# Autodesk Inventor assembly: Z Rail Right
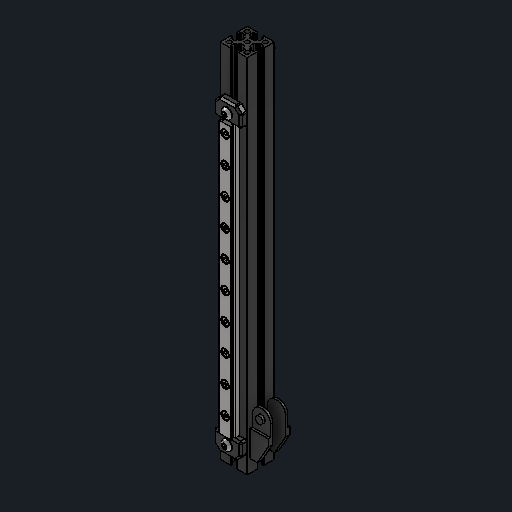
[picture p0: Inventor's stored thumbnail of the model, 512x512]
Saved by Autodesk Inventor 2026.1 (Build 301233020, 233B)
## iProperties
Created: 2025-05-11
Part Number: Z Rail Right
Document SubType Name: Assembly
Designer: Joshua Eah
Author: Joshua Eah
## Documents named in this file (9)
- C:\Users\JoshuaEah\Documents\GitHub\Voron-0\CAD\Z Axis\Z Extrusion Right.iam
- Z Extrusion Right.iam
- C:\Users\JoshuaEah\Documents\GitHub\Voron-0\CAD\Frame\Parts\1515_200mm - C.ipt
- C:\Users\JoshuaEah\Documents\GitHub\Voron-0\CAD\Hardware\M3x6 BHCS.ipt
- C:\Users\JoshuaEah\Documents\GitHub\Voron-0\CAD\Hardware\M3 Hexnut.ipt
- C:\Users\JoshuaEah\Documents\GitHub\Voron-0\CAD\Linear Rail\MGN7 Rail 150mm.iam
- MGN7 150mm Rail.iam
- C:\Users\JoshuaEah\Documents\GitHub\Voron-0\CAD\Frame\Subassemblies\Rail Stop.iam
- C:\Users\JoshuaEah\Documents\GitHub\Voron-0\CAD\Z Axis\Subassemblies\Chain Link End.iam
## Components (9 placed, 6 different names)
1. 1515_200mm - C:1
2. MGN7 Rail 150mm:1 [sub-assembly]
3. Rail Stop:1 [sub-assembly]
4. Rail Stop:2 [sub-assembly]
5. Chain Link End:1 [sub-assembly]
6. M3x6 BHCS:1
7. M3x6 BHCS:2
8. M3 Hexnut:1
9. M3 Hexnut:2
## Relationships (17: Mate 11, Flush 4, Insert 2)
- [Mate]: 1515_200mm - C:1 ↔ M3x6 BHCS:1
- [Mate]: 1515_200mm - C:1 ↔ M3x6 BHCS:1
- [Insert]: M3x6 BHCS:1 ↔ M3 Hexnut:1
- [Mate]: 1515_200mm - C:1 ↔ M3x6 BHCS:2
- [Mate]: 1515_200mm - C:1 ↔ M3x6 BHCS:2
- [Insert]: M3x6 BHCS:2 ↔ M3 Hexnut:2
- [Mate]: 1515_200mm - C:1 ↔ MGN7 Rail 150mm:1
- [Flush] (33 mm): 1515_200mm - C:1 ↔ MGN7 Rail 150mm:1
- [Mate] (0.1 mm): 1515_200mm - C:1 ↔ MGN7 Rail 150mm:1
- [Mate]: 1515_200mm - C:1 ↔ Rail Stop:1
- [Mate]: MGN7 Rail 150mm:1 ↔ Rail Stop:1
- [Flush]: 1515_200mm - C:1 ↔ Rail Stop:1
- [Mate]: MGN7 Rail 150mm:1 ↔ Rail Stop:2
- [Mate]: 1515_200mm - C:1 ↔ Rail Stop:2
- [Flush]: 1515_200mm - C:1 ↔ Rail Stop:2
- [Flush]: Rail Stop:2 ↔ Chain Link End:1
- [Mate]: 1515_200mm - C:1 ↔ Chain Link End:1
## Named parameters: d9_d12 = 33 mm, d14_d19 = 0 mm, d16_d20 = 0 mm
